# Autodesk Inventor assembly: liftPose_device
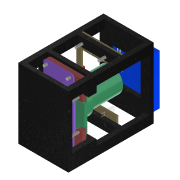
[picture p0: Inventor's stored thumbnail of the model, 180x180]
Saved by Autodesk Inventor 2021 (Build 250183000, 183)
## iProperties
Created: 2021-02-15
Part Number: liftPose_device
Document SubType Name: Assembly
Designer: lobato
Author: lobato
## Documents named in this file (7)
- C:\Users\lobato\Desktop\LiftPose3d-device\v2_raspberry\liftPose_device.iam
- C:\Users\lobato\Desktop\LiftPose3d-device\v2_raspberry\camera_module.iam
- C:\Users\lobato\Desktop\LiftPose3d-device\v2_raspberry\arena_top_bottom.ipt
- C:\Users\lobato\Desktop\LiftPose3d-device\v2_raspberry\arena_middle.ipt
- C:\Users\lobato\Desktop\LiftPose3d-device\v2_raspberry\circuit\circuit.iam
- C:\Users\lobato\Desktop\LiftPose3d-device\v2_raspberry\screwM2-5.ipt
- C:\Users\lobato\Desktop\LiftPose3d-device\v2_raspberry\base.ipt
## Components (15 placed, 6 different names)
1. camera_module:1 [sub-assembly] — Insert:15, Insert:16, Insert:22, Insert:23
2. arena_top_bottom:1 — Insert:4, Insert:17, Insert:18, Insert:19
3. arena_middle:1 — Insert:4, Insert:5, Insert:19
4. arena_top_bottom:2 — Insert:5
5. circuit:1 [sub-assembly] — Insert:8, Insert:9, Insert:10, Insert:20, Insert:21
6. screwM2-5:1 — Insert:27
7. screwM2-5:2 — Insert:26
8. screwM2-5:3 — Insert:24
9. screwM2-5:4 — Insert:9
10. screwM2-5:5 — Insert:16
11. screwM2-5:6 — Insert:15
12. screwM2-5:7 — Insert:10
13. screwM2-5:8 — Insert:8
14. screwM2-5:9 — Insert:25
15. base:1 — Insert:17, Insert:18, Insert:20, Insert:21, Insert:22, Insert:23, Insert:24, Insert:25, Insert:26, Insert:27
## Relationships (18: Insert 18)
- Insert:4: arena_top_bottom:1 ↔ arena_middle:1
- Insert:5: arena_middle:1 ↔ arena_top_bottom:2
- Insert:8: circuit:1 ↔ screwM2-5:8
- Insert:9: circuit:1 ↔ screwM2-5:4
- Insert:10: circuit:1 ↔ screwM2-5:7
- Insert:15: camera_module:1 ↔ screwM2-5:6
- Insert:16: camera_module:1 ↔ screwM2-5:5
- Insert:17: arena_top_bottom:1 ↔ base:1
- Insert:18: arena_top_bottom:1 ↔ base:1
- Insert:19: arena_top_bottom:1 ↔ arena_middle:1
- Insert:20: circuit:1 ↔ base:1
- Insert:21: circuit:1 ↔ base:1
- Insert:22: camera_module:1 ↔ base:1
- Insert:23: camera_module:1 ↔ base:1
- Insert:24: screwM2-5:3 ↔ base:1
- Insert:25: screwM2-5:9 ↔ base:1
- Insert:26: screwM2-5:2 ↔ base:1
- Insert:27: screwM2-5:1 ↔ base:1
